# Autodesk Inventor assembly: SandTimer
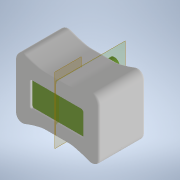
[picture p0: Inventor's stored thumbnail of the model, 180x180]
Saved by Autodesk Inventor 2021 (Build 250183000, 183)
## iProperties
Created: 2023-12-26
Part Number: SandTimer
Document SubType Name: Assembly
Designer: maxsm
Author: maxsm
## Documents named in this file (4)
- C:\Users\maxsm\root\SandTimer\casings\SandTimer.iam
- C:\Users\maxsm\root\SandTimer\casings\Electronic Assembly.ipt
- C:\Users\maxsm\root\SandTimer\casings\FrontCasing.ipt
- C:\Users\maxsm\root\SandTimer\casings\BackCasing.ipt
## Components (3 placed, 3 different names)
1. Electronic Assembly:1 — Mate:1, Mate:2, Mate:6
2. FrontCasing:1 — Mate:1, Mate:2, Mate:3, Mate:4, Mate:5, Mate:6
3. BackCasing:1 — Mate:3, Mate:4, Mate:5
## Relationships (6: Mate 6)
- Mate:1: Electronic Assembly:1 ↔ FrontCasing:1
- Mate:2: Electronic Assembly:1 ↔ FrontCasing:1
- Mate:3: FrontCasing:1 ↔ BackCasing:1
- Mate:4: FrontCasing:1 ↔ BackCasing:1
- Mate:5: FrontCasing:1 ↔ BackCasing:1
- Mate:6: Electronic Assembly:1 ↔ FrontCasing:1
